# Autodesk Inventor assembly: TKS ASY Mixer frame
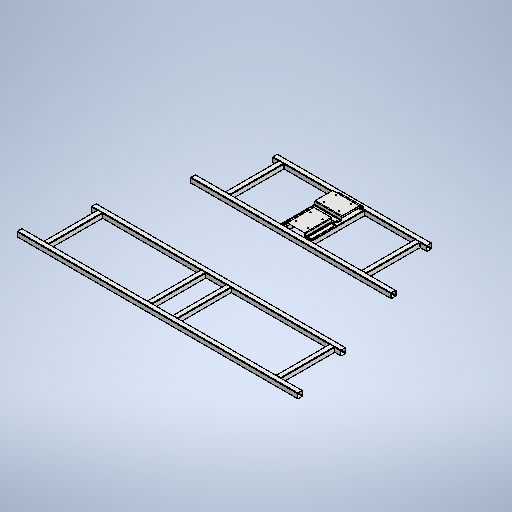
[picture p0: Inventor's stored thumbnail of the model, 512x512]
Saved by Autodesk Inventor 2025.3 (Build 293356030, 356C)
## iProperties
_SolveAssemblyDoc: Frame Generator Solve Assembly
_Version: 25.0.0
Created: 2025-08-15
Part Number: TKS ASY Mixer frame
Document SubType Name: Assembly
Designer: admin
Author: admin
## Documents named in this file (4)
- C:\Users\admin\Yandex.Disk\home pc\Inventor\TKS-Tarko-Sale\TKS ASY Mixer frame.iam
- C:\Users\admin\Yandex.Disk\home pc\Inventor\TKS-Tarko-Sale\TKS mixer frame sketch.ipt
- C:\Users\admin\Yandex.Disk\home pc\Inventor\TKS-Tarko-Sale\TKS ASY Mixer frame\Frame\Frame 1755240995115.iam
- C:\Users\admin\Yandex.Disk\home pc\Inventor\TKS-Tarko-Sale\TKS mixer support.ipt
## Components (4 placed, 3 different names)
1. TKS mixer frame sketch:1
2. Frame 1755240995115:1 [sub-assembly] — Mate:1, Mate:3
3. TKS mixer support:1 — Mate:1
4. TKS mixer support:2 — Mate:3
## Relationships (2: Mate 2)
- Mate:1: Frame 1755240995115:1 ↔ TKS mixer support:1
- Mate:3: Frame 1755240995115:1 ↔ TKS mixer support:2
